# Autodesk Inventor assembly: capsule.bottom.assembly
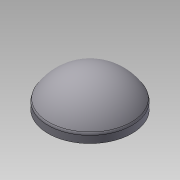
[picture p0: Inventor's stored thumbnail of the model, 180x180]
Saved by Autodesk Inventor 2011 (Build 150239000, 239)
## iProperties
Created: 2011-01-27
Part Number: capsule.bottom.assembly
Document SubType Name: Assembly
Designer: Casey
Author: Casey
## Documents named in this file (6)
- C:\Users\M. Woods III\Desktop\design\Mechanical Drawings\capsule_bottom.iam
- C:\Users\M. Woods III\Desktop\design\Mechanical Drawings\capsule_bottom.ipt
- C:\Users\M. Woods III\Desktop\design\Mechanical Drawings\capsule_electronics.ipt
- C:\Users\M. Woods III\Desktop\design\Mechanical Drawings\capsule_gasket.ipt
- C:\Users\M. Woods III\Desktop\design\Mechanical Drawings\elecbox_3mm-standoff-16-long.ipt
- C:\Users\M. Woods III\Desktop\design\Mechanical Drawings\ANSI B18.3.1M(6)\ANSI B18.3.1M - M3x0.5 x 5(1).ipt
## Components (16 placed, 5 different names)
1. capsule_bottom:1 — Mate:1, Mate:2, Mate:3, Mate:4, Mate:5, Mate:6, Mate:7
2. capsule_electronics:1 — Mate:1, Mate:2, Mate:3, Insert:1
3. capsule_gasket:1 — Mate:4, Mate:5, Mate:6
4. capsule_electronics:2 — Mate:7, Mate:8, Mate:9, Insert:2, Insert:3, Insert:4, Insert:5, Insert:6, Insert:7
5. Forged Socket Head Cap Screw - Metric M3x0.5 x 5:1 — Insert:2
6. Forged Socket Head Cap Screw - Metric M3x0.5 x 5:2 — Insert:3
7. Forged Socket Head Cap Screw - Metric M3x0.5 x 5:3 — Insert:4
8. Forged Socket Head Cap Screw - Metric M3x0.5 x 5:4 — Insert:5
9. Forged Socket Head Cap Screw - Metric M3x0.5 x 5:5 — Insert:6
10. Forged Socket Head Cap Screw - Metric M3x0.5 x 5:6 — Insert:7
11. elecbox_3mm-standoff-16-long:1 — Insert:1
12. elecbox_3mm-standoff-16-long:2
13. elecbox_3mm-standoff-16-long:3
14. elecbox_3mm-standoff-16-long:4
15. elecbox_3mm-standoff-16-long:5
16. elecbox_3mm-standoff-16-long:6 — Mate:8, Mate:9
## Component patterns: (6 elements, first: elecbox_3mm-standoff-16-long:1)
## Relationships (16: Mate 9, Insert 7)
- Mate:1: capsule_bottom:1 ↔ capsule_electronics:1
- Mate:2: capsule_bottom:1 ↔ capsule_electronics:1
- Mate:3: capsule_bottom:1 ↔ capsule_electronics:1
- Mate:4: capsule_bottom:1 ↔ capsule_gasket:1
- Mate:5: capsule_bottom:1 ↔ capsule_gasket:1
- Mate:6: capsule_bottom:1 ↔ capsule_gasket:1
- Insert:1: capsule_electronics:1 ↔ elecbox_3mm-standoff-16-long:1
- Mate:7: capsule_bottom:1 ↔ capsule_electronics:2
- Mate:8: capsule_electronics:2 ↔ elecbox_3mm-standoff-16-long:6
- Mate:9: capsule_electronics:2 ↔ elecbox_3mm-standoff-16-long:6
- Insert:2: capsule_electronics:2 ↔ Forged Socket Head Cap Screw - Metric M3x0.5 x 5:1
- Insert:3: capsule_electronics:2 ↔ Forged Socket Head Cap Screw - Metric M3x0.5 x 5:2
- Insert:4: capsule_electronics:2 ↔ Forged Socket Head Cap Screw - Metric M3x0.5 x 5:3
- Insert:5: capsule_electronics:2 ↔ Forged Socket Head Cap Screw - Metric M3x0.5 x 5:4
- Insert:6: capsule_electronics:2 ↔ Forged Socket Head Cap Screw - Metric M3x0.5 x 5:5
- Insert:7: capsule_electronics:2 ↔ Forged Socket Head Cap Screw - Metric M3x0.5 x 5:6
